# Autodesk Inventor assembly: Plasma-vacuum-vessel-34IC-cross
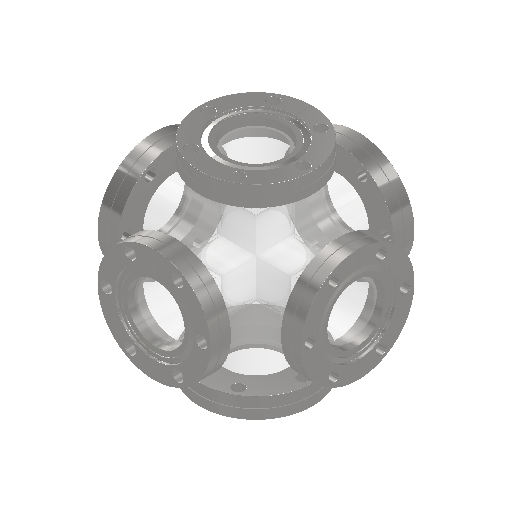
[picture p0: Inventor's stored thumbnail of the model, 512x512]
Saved by Autodesk Inventor 2026.2 (Build 302298000, 298)
## iProperties
Created: 2024-01-30
Part Number: Plasma-vacuum-vessel-34IC-cross
Document SubType Name: Assembly
Designer: zetsu
Sending System: Autodesk Inventor 2024
Preprocessor: ST-DEVELOPER v19.2
Title: ICF70SWX.stp
Author: Part-time7
## Documents named in this file (3)
- D:\repos\PIHTI\Plasma Vessel_2026\Plasma-vacuum-vessel\Plasma-vacuum-vessel-34IC-cross.iam
- D:\repos\PIHTI\Plasma Vessel_2026\Plasma-vacuum-vessel\Cross-6way-34IC.ipt
- D:\repos\PIHTI\Plasma Vessel_2026\Plasma-vacuum-vessel\UFC-34.ipt
## Components (7 placed, 2 different names)
1. Cross-6way-34IC:1 — リジッド:1, リジッド:2, リジッド:3, リジッド:4, リジッド:5, リジッド:6
2. UFC-34:1 — リジッド:1
3. UFC-34:2 — リジッド:2
4. UFC-34:3 — リジッド:3
5. UFC-34:4 — リジッド:4
6. UFC-34:5 — リジッド:5
7. UFC-34:6 — リジッド:6
## Relationships (6: WeldJoint 6)
- リジッド:1 [WeldJoint]: Cross-6way-34IC:1 ↔ UFC-34:1
- リジッド:2 [WeldJoint]: Cross-6way-34IC:1 ↔ UFC-34:2
- リジッド:3 [WeldJoint]: Cross-6way-34IC:1 ↔ UFC-34:3
- リジッド:4 [WeldJoint]: Cross-6way-34IC:1 ↔ UFC-34:4
- リジッド:5 [WeldJoint]: Cross-6way-34IC:1 ↔ UFC-34:5
- リジッド:6 [WeldJoint]: Cross-6way-34IC:1 ↔ UFC-34:6
